# Autodesk Inventor assembly: 42146-21
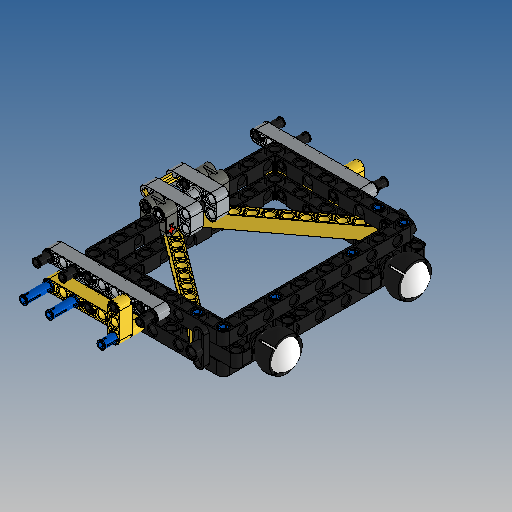
[picture p0: Inventor's stored thumbnail of the model, 512x512]
Saved by Autodesk Inventor 2025 (Build 290162010, 162A)
## iProperties
Created: 2024-11-22
Part Number: 42146-21
Material: Generisch
Document SubType Name: Assembly
Designer: hp.muther
Author: hp.muther
## Documents named in this file (17)
- D:\Inventor\Projekte\Muther\LEGO Technic\LEGO Technik - Raupenkran LR 13000 (42146)\42146-21.iam
- D:\Inventor\Projekte\Muther\LEGO Technic\LEGO Pieces\Rahmen, T-Stücke\39790-Black.ipt
- D:\Inventor\Projekte\Muther\LEGO Technic\LEGO Pieces\Pin's\2780-Black.ipt
- D:\Inventor\Projekte\Muther\LEGO Technic\LEGO Pieces\Pin's\11214-Red.ipt
- D:\Inventor\Projekte\Muther\LEGO Technic\LEGO Pieces\Pin's\32054-LtBluishGray.ipt
- D:\Inventor\Projekte\Muther\LEGO Technic\LEGO Pieces\Pin's\6558-Blue.ipt
- D:\Inventor\Projekte\Muther\LEGO Technic\LEGO Pieces\Achsen\4519-Yellow.ipt
- D:\Inventor\Projekte\Muther\LEGO Technic\LEGO Pieces\Achsen\32062-Red.ipt
- D:\Inventor\Projekte\Muther\LEGO Technic\LEGO Pieces\Winkel\32140-LtBluishGray.ipt
- D:\Inventor\Projekte\Muther\LEGO Technic\LEGO Pieces\Verbindungselemente\41678-DkBluishGray.ipt
- D:\Inventor\Projekte\Muther\LEGO Technic\LEGO Pieces\Lochbalken\40490-LtBluishGray.ipt
- D:\Inventor\Projekte\Muther\LEGO Technic\LEGO Pieces\Lochbalken\32525-Yellow.ipt
- D:\Inventor\Projekte\Muther\LEGO Technic\LEGO Pieces\Lochbalken\32524-Yellow.ipt
- D:\Inventor\Projekte\Muther\LEGO Technic\LEGO Pieces\Lochbalken\32523-Yellow.ipt
- D:\Inventor\Projekte\Muther\LEGO Technic\LEGO Pieces\Verbindungselemente\15461-Black.ipt
- D:\Inventor\Projekte\Muther\LEGO Technic\LEGO Pieces\Diverses\39370-Black.ipt
- D:\Inventor\Projekte\Muther\LEGO Technic\LEGO Pieces\Diverses\52629-White.ipt
## Components (57 placed, 16 different names)
1. 39790-Black:1 — Passend:4, Passend:5, Passend:6, Einfügen:23, Einfügen:24, Passend:7, Passend:8, Einfügen:25, Einfügen:26, Einfügen:27, Einfügen:28, Einfügen:29, Einfügen:30, Einfügen:50, Einfügen:51
2. 2780-Black:1 — Einfügen:16, Passend:2
3. 11214-Red:1 — Einfügen:17, Einfügen:20
4. 32054-LtBluishGray:1 — Einfügen:17, Einfügen:18
5. 2780-Black:2 — Einfügen:19, Passend:3
6. 2780-Black:3 — Einfügen:3
7. 2780-Black:4 — Einfügen:4
8. 2780-Black:5 — Einfügen:5
9. 2780-Black:6 — Einfügen:6
10. 2780-Black:7 — Einfügen:8
11. 2780-Black:8 — Einfügen:7, Passend:7
12. 6558-Blue:1 — Einfügen:31
13. 6558-Blue:2 — Einfügen:32, Passend:18
14. 6558-Blue:3 — Einfügen:34
15. 6558-Blue:4 — Einfügen:33, Passend:19
16. 6558-Blue:5 — Einfügen:26, Passend:11
17. 6558-Blue:6 — Einfügen:28, Passend:9
18. 6558-Blue:7 — Einfügen:27, Passend:10
19. 6558-Blue:8 — Einfügen:25
20. 4519-Yellow:1 — Einfügen:15
21. 32062-Red:1 — Einfügen:1, Passend:5
22. 32140-LtBluishGray:1 — Einfügen:15, Einfügen:16, Einfügen:18, Passend:1, Einfügen:22
23. 32140-LtBluishGray:2 — Einfügen:19, Einfügen:20, Passend:1, Einfügen:21
24. 41678-DkBluishGray:1 — Einfügen:1, Einfügen:22, Passend:2
25. 32062-Red:2 — Passend:4
26. 41678-DkBluishGray:2 — Einfügen:21, Passend:3, Passend:6
27. 40490-LtBluishGray:1 — Einfügen:3, Einfügen:4, Einfügen:5, Einfügen:6, Einfügen:7, Einfügen:8, Einfügen:23, Einfügen:48
28. 2780-Black:9
29. 2780-Black:10
30. 2780-Black:11
31. 2780-Black:12
32. 2780-Black:13
33. 2780-Black:14 — Passend:8
34. 40490-LtBluishGray:2 — Einfügen:24, Einfügen:49
35. 32525-Yellow:1 — Einfügen:29, Passend:9, Einfügen:35
36. 32525-Yellow:2 — Einfügen:30, Passend:10
37. 39790-Black:2 — Einfügen:31, Einfügen:32, Einfügen:33, Einfügen:34, Einfügen:35, Passend:11, Einfügen:46, Einfügen:47, Passend:12, Passend:13, Einfügen:52, Passend:16, Einfügen:53, Einfügen:54
38. 32524-Yellow:1 — Einfügen:36, Einfügen:37, Einfügen:38, Einfügen:39, Einfügen:40, Einfügen:46
39. 6558-Blue:9 — Einfügen:36
40. 6558-Blue:10 — Einfügen:37
41. 6558-Blue:11 — Einfügen:38, Passend:15
42. 2780-Black:15 — Einfügen:39
43. 2780-Black:16 — Einfügen:40, Passend:13
44. 32524-Yellow:2 — Einfügen:47
45. 6558-Blue:12
46. 6558-Blue:13
47. 6558-Blue:14 — Passend:14
48. 2780-Black:17
49. 2780-Black:18 — Passend:12
50. 32523-Yellow:1 — Einfügen:48, Passend:15
51. 32523-Yellow:2 — Einfügen:49, Passend:14
52. 15461-Black:1 — Einfügen:50, Passend:16
53. 15461-Black:2 — Einfügen:51, Einfügen:52
54. 39370-Black:1 — Passend:17, Passend:18, Einfügen:54
55. 52629-White:1 — Passend:17
56. 39370-Black:2 — Passend:19, Einfügen:53, Passend:20
57. 52629-White:2 — Passend:20
## Relationships (74: Insert 54, Mate 20)
- Einfügen:1 [Insert]: 32062-Red:1 ↔ 41678-DkBluishGray:1
- [Insert]: 32062-Red:2 ↔ 41678-DkBluishGray:2
- Einfügen:3 [Insert]: 2780-Black:3 ↔ 40490-LtBluishGray:1
- Einfügen:4 [Insert]: 2780-Black:4 ↔ 40490-LtBluishGray:1
- Einfügen:5 [Insert]: 2780-Black:5 ↔ 40490-LtBluishGray:1
- Einfügen:6 [Insert]: 2780-Black:6 ↔ 40490-LtBluishGray:1
- Einfügen:7 [Insert]: 2780-Black:8 ↔ 40490-LtBluishGray:1
- Einfügen:8 [Insert]: 2780-Black:7 ↔ 40490-LtBluishGray:1
- [Insert]: 2780-Black:9 ↔ 40490-LtBluishGray:2
- [Insert]: 2780-Black:10 ↔ 40490-LtBluishGray:2
- [Insert]: 2780-Black:11 ↔ 40490-LtBluishGray:2
- [Insert]: 2780-Black:12 ↔ 40490-LtBluishGray:2
- [Insert]: 2780-Black:14 ↔ 40490-LtBluishGray:2
- [Insert]: 2780-Black:13 ↔ 40490-LtBluishGray:2
- Einfügen:15 [Insert]: 4519-Yellow:1 ↔ 32140-LtBluishGray:1
- Einfügen:16 [Insert]: 2780-Black:1 ↔ 32140-LtBluishGray:1
- Einfügen:17 [Insert]: 11214-Red:1 ↔ 32054-LtBluishGray:1
- Einfügen:18 [Insert]: 32054-LtBluishGray:1 ↔ 32140-LtBluishGray:1
- Einfügen:19 [Insert]: 2780-Black:2 ↔ 32140-LtBluishGray:2
- Einfügen:20 [Insert]: 11214-Red:1 ↔ 32140-LtBluishGray:2
- Passend:1 [Mate]: 32140-LtBluishGray:1 ↔ 32140-LtBluishGray:2
- Einfügen:21 [Insert]: 32140-LtBluishGray:2 ↔ 41678-DkBluishGray:2
- Einfügen:22 [Insert]: 32140-LtBluishGray:1 ↔ 41678-DkBluishGray:1
- Passend:2 [Mate]: 2780-Black:1 ↔ 41678-DkBluishGray:1
- Passend:3 [Mate]: 2780-Black:2 ↔ 41678-DkBluishGray:2
- Passend:4 [Mate]: 39790-Black:1 ↔ 32062-Red:2
- Passend:5 [Mate]: 39790-Black:1 ↔ 32062-Red:1
- Passend:6 [Mate]: 39790-Black:1 ↔ 41678-DkBluishGray:2
- Einfügen:23 [Insert]: 39790-Black:1 ↔ 40490-LtBluishGray:1
- Einfügen:24 [Insert]: 39790-Black:1 ↔ 40490-LtBluishGray:2
- Passend:7 [Mate]: 39790-Black:1 ↔ 2780-Black:8
- Passend:8 [Mate]: 39790-Black:1 ↔ 2780-Black:14
- Einfügen:25 [Insert]: 39790-Black:1 ↔ 6558-Blue:8
- Einfügen:26 [Insert]: 39790-Black:1 ↔ 6558-Blue:5
- Einfügen:27 [Insert]: 39790-Black:1 ↔ 6558-Blue:7
- Einfügen:28 [Insert]: 39790-Black:1 ↔ 6558-Blue:6
- Einfügen:29 [Insert]: 39790-Black:1 ↔ 32525-Yellow:1
- Einfügen:30 [Insert]: 39790-Black:1 ↔ 32525-Yellow:2
- Passend:9 [Mate]: 6558-Blue:6 ↔ 32525-Yellow:1
- Passend:10 [Mate]: 6558-Blue:7 ↔ 32525-Yellow:2
- Einfügen:31 [Insert]: 6558-Blue:1 ↔ 39790-Black:2
- Einfügen:32 [Insert]: 6558-Blue:2 ↔ 39790-Black:2
- Einfügen:33 [Insert]: 6558-Blue:4 ↔ 39790-Black:2
- Einfügen:34 [Insert]: 6558-Blue:3 ↔ 39790-Black:2
- Einfügen:35 [Insert]: 32525-Yellow:1 ↔ 39790-Black:2
- Passend:11 [Mate]: 6558-Blue:5 ↔ 39790-Black:2
- Einfügen:36 [Insert]: 32524-Yellow:1 ↔ 6558-Blue:9
- Einfügen:37 [Insert]: 32524-Yellow:1 ↔ 6558-Blue:10
- Einfügen:38 [Insert]: 32524-Yellow:1 ↔ 6558-Blue:11
- Einfügen:39 [Insert]: 32524-Yellow:1 ↔ 2780-Black:15
- Einfügen:40 [Insert]: 32524-Yellow:1 ↔ 2780-Black:16
- [Insert]: 32524-Yellow:2 ↔ 6558-Blue:12
- [Insert]: 32524-Yellow:2 ↔ 6558-Blue:13
- [Insert]: 32524-Yellow:2 ↔ 6558-Blue:14
- [Insert]: 32524-Yellow:2 ↔ 2780-Black:17
- [Insert]: 32524-Yellow:2 ↔ 2780-Black:18
- Einfügen:46 [Insert]: 39790-Black:2 ↔ 32524-Yellow:1
- Einfügen:47 [Insert]: 39790-Black:2 ↔ 32524-Yellow:2
- Passend:12 [Mate]: 39790-Black:2 ↔ 2780-Black:18
- Passend:13 [Mate]: 39790-Black:2 ↔ 2780-Black:16
- Einfügen:48 [Insert]: 40490-LtBluishGray:1 ↔ 32523-Yellow:1
- Einfügen:49 [Insert]: 40490-LtBluishGray:2 ↔ 32523-Yellow:2
- Passend:14 [Mate]: 6558-Blue:14 ↔ 32523-Yellow:2
- Passend:15 [Mate]: 6558-Blue:11 ↔ 32523-Yellow:1
- Einfügen:50 [Insert]: 39790-Black:1 ↔ 15461-Black:1
- Einfügen:51 [Insert]: 39790-Black:1 ↔ 15461-Black:2
- Einfügen:52 [Insert]: 39790-Black:2 ↔ 15461-Black:2
- Passend:16 [Mate]: 39790-Black:2 ↔ 15461-Black:1
- Passend:17 [Mate]: 39370-Black:1 ↔ 52629-White:1
- Passend:18 [Mate]: 6558-Blue:2 ↔ 39370-Black:1
- Passend:19 [Mate]: 6558-Blue:4 ↔ 39370-Black:2
- Einfügen:53 [Insert]: 39790-Black:2 ↔ 39370-Black:2
- Einfügen:54 [Insert]: 39790-Black:2 ↔ 39370-Black:1
- Passend:20 [Mate]: 39370-Black:2 ↔ 52629-White:2
## Named parameters: d1_d0 = 0 mm, d8_d2 = 0 mm, d9_d3 = 0 mm, d10_d4 = 0 mm, d11_d5 = 0 mm, d12_d6 = 0 mm, d13_d7 = 0 mm, d51_d50 = 0 mm, d52_d46 = 0 mm, d53_d47 = 0 mm, d54_d48 = 0 mm, d55_d49 = 0 mm
